# Autodesk Inventor assembly: PCBDiplomPCB
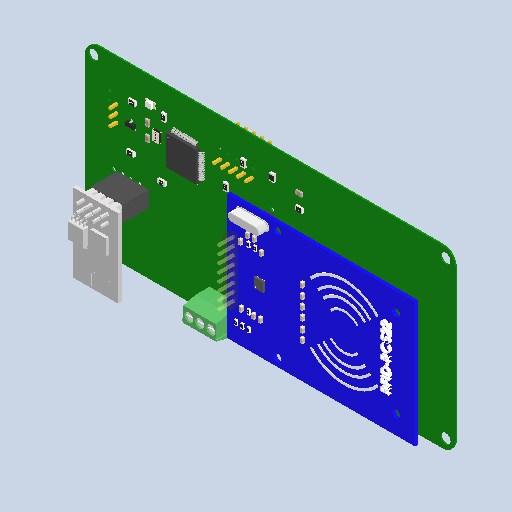
[picture p0: Inventor's stored thumbnail of the model, 512x512]
Saved by Autodesk Inventor 2022 (Build 260153000, 153)
## iProperties
Company: Open CASCADE
Created: 2022-05-22
Part Number: PCBDiplomPCB
Description: Open CASCADE Model
Document SubType Name: Assembly
Designer: user
Authority: Unknown
Sending System: Open CASCADE 6.8
Preprocessor: Open CASCADE STEP processor 6.8
Title: Open CASCADE Shape Model
Author: Author
## Documents named in this file (45)
- C:\Study\Diplom\Altium\Diplom\Project Outputs for Diplom\InventorNew\PCBDiplomPCB.iam
- C:\Study\Diplom\Altium\Diplom\Project Outputs for Diplom\InventorNew\PCBBoard.iam
- C:\Study\Diplom\Altium\Diplom\Project Outputs for Diplom\InventorNew\PCBDA1.iam
- C:\Study\Diplom\Altium\Diplom\Project Outputs for Diplom\InventorNew\PCBR14.iam
- C:\Study\Diplom\Altium\Diplom\Project Outputs for Diplom\InventorNew\PCBR13.iam
- C:\Study\Diplom\Altium\Diplom\Project Outputs for Diplom\InventorNew\PCBR11.iam
- C:\Study\Diplom\Altium\Diplom\Project Outputs for Diplom\InventorNew\PCBR6.iam
- C:\Study\Diplom\Altium\Diplom\Project Outputs for Diplom\InventorNew\PCBR5.iam
- C:\Study\Diplom\Altium\Diplom\Project Outputs for Diplom\InventorNew\PCBR4.iam
- C:\Study\Diplom\Altium\Diplom\Project Outputs for Diplom\InventorNew\PCBR3.iam
- C:\Study\Diplom\Altium\Diplom\Project Outputs for Diplom\InventorNew\PCBZQ1.iam
- C:\Study\Diplom\Altium\Diplom\Project Outputs for Diplom\InventorNew\PCBXS4.iam
- C:\Study\Diplom\Altium\Diplom\Project Outputs for Diplom\InventorNew\PCBXS3.iam
- C:\Study\Diplom\Altium\Diplom\Project Outputs for Diplom\InventorNew\PCBXS2.iam
- C:\Study\Diplom\Altium\Diplom\Project Outputs for Diplom\InventorNew\PCBXS1.iam
- C:\Study\Diplom\Altium\Diplom\Project Outputs for Diplom\InventorNew\PCBXP2.iam
- C:\Study\Diplom\Altium\Diplom\Project Outputs for Diplom\InventorNew\PCBXP1.iam
- C:\Study\Diplom\Altium\Diplom\Project Outputs for Diplom\InventorNew\PCBVT1.iam
- C:\Study\Diplom\Altium\Diplom\Project Outputs for Diplom\InventorNew\PCBSB1.iam
- C:\Study\Diplom\Altium\Diplom\Project Outputs for Diplom\InventorNew\PCBSA1.iam
- C:\Study\Diplom\Altium\Diplom\Project Outputs for Diplom\InventorNew\PCBR12.iam
- C:\Study\Diplom\Altium\Diplom\Project Outputs for Diplom\InventorNew\PCBR8.iam
- C:\Study\Diplom\Altium\Diplom\Project Outputs for Diplom\InventorNew\PCBR7.iam
- C:\Study\Diplom\Altium\Diplom\Project Outputs for Diplom\InventorNew\PCBR10.iam
- C:\Study\Diplom\Altium\Diplom\Project Outputs for Diplom\InventorNew\PCBR9.iam
- C:\Study\Diplom\Altium\Diplom\Project Outputs for Diplom\InventorNew\PCBR2.iam
- C:\Study\Diplom\Altium\Diplom\Project Outputs for Diplom\InventorNew\PCBR1.iam
- C:\Study\Diplom\Altium\Diplom\Project Outputs for Diplom\InventorNew\PCBL1.iam
- C:\Study\Diplom\Altium\Diplom\Project Outputs for Diplom\InventorNew\PCBHL1.iam
- C:\Study\Diplom\Altium\Diplom\Project Outputs for Diplom\InventorNew\PCBF1.iam
- C:\Study\Diplom\Altium\Diplom\Project Outputs for Diplom\InventorNew\PCBDD1.iam
- C:\Study\Diplom\Altium\Diplom\Project Outputs for Diplom\InventorNew\PCBC14.iam
- C:\Study\Diplom\Altium\Diplom\Project Outputs for Diplom\InventorNew\PCBC13.iam
- C:\Study\Diplom\Altium\Diplom\Project Outputs for Diplom\InventorNew\PCBC12.iam
- C:\Study\Diplom\Altium\Diplom\Project Outputs for Diplom\InventorNew\PCBC11.iam
- C:\Study\Diplom\Altium\Diplom\Project Outputs for Diplom\InventorNew\PCBC10.iam
- C:\Study\Diplom\Altium\Diplom\Project Outputs for Diplom\InventorNew\PCBC9.iam
- C:\Study\Diplom\Altium\Diplom\Project Outputs for Diplom\InventorNew\PCBC8.iam
- C:\Study\Diplom\Altium\Diplom\Project Outputs for Diplom\InventorNew\PCBC7.iam
- C:\Study\Diplom\Altium\Diplom\Project Outputs for Diplom\InventorNew\PCBC6.iam
- C:\Study\Diplom\Altium\Diplom\Project Outputs for Diplom\InventorNew\PCBC5.iam
- C:\Study\Diplom\Altium\Diplom\Project Outputs for Diplom\InventorNew\PCBC4.iam
- C:\Study\Diplom\Altium\Diplom\Project Outputs for Diplom\InventorNew\PCBC3.iam
- C:\Study\Diplom\Altium\Diplom\Project Outputs for Diplom\InventorNew\PCBC2.iam
- C:\Study\Diplom\Altium\Diplom\Project Outputs for Diplom\InventorNew\PCBC1.iam
## Components (44 placed, 44 different names)
1. Board_2 [sub-assembly] — Совмещение:1, Совмещение:2
2. DA1_4 [sub-assembly]
3. R14_6 [sub-assembly]
4. R13_8 [sub-assembly]
5. R11_10 [sub-assembly]
6. R6_12 [sub-assembly]
7. R5_14 [sub-assembly]
8. R4_16 [sub-assembly]
9. R3_18 [sub-assembly]
10. ZQ1_20 [sub-assembly]
11. XS4_22 [sub-assembly] — Совмещение:1, Совмещение:2
12. XS3_48 [sub-assembly]
13. XS2_64 [sub-assembly]
14. XS1_66 [sub-assembly]
15. XP2_70 [sub-assembly]
16. XP1_76 [sub-assembly]
17. VT1_78 [sub-assembly]
18. SB1_80 [sub-assembly]
19. SA1_83 [sub-assembly]
20. R12_85 [sub-assembly]
21. R8_87 [sub-assembly]
22. R7_89 [sub-assembly]
23. R10_91 [sub-assembly]
24. R9_93 [sub-assembly]
25. R2_95 [sub-assembly]
26. R1_97 [sub-assembly]
27. L1_102 [sub-assembly]
28. HL1_104 [sub-assembly]
29. F1_106 [sub-assembly]
30. DD1_108 [sub-assembly]
31. C14_110 [sub-assembly]
32. C13_112 [sub-assembly]
33. C12_114 [sub-assembly]
34. C11_116 [sub-assembly]
35. C10_118 [sub-assembly]
36. C9_120 [sub-assembly]
37. C8_122 [sub-assembly]
38. C7_124 [sub-assembly]
39. C6_126 [sub-assembly]
40. C5_128 [sub-assembly]
41. C4_130 [sub-assembly]
42. C3_132 [sub-assembly]
43. C2_134 [sub-assembly]
44. C1_136 [sub-assembly]
## Relationships (2: Mate 2)
- Совмещение:1 [Mate]: Board_2 ↔ XS4_22
- Совмещение:2 [Mate]: Board_2 ↔ XS4_22
